# Autodesk Inventor assembly: Aluminium profile system
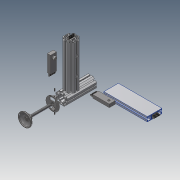
[picture p0: Inventor's stored thumbnail of the model, 180x180]
Saved by Autodesk Inventor 2015 (Build 190159000, 159)
## iProperties
Created: 2016-03-14
Part Number: Aluminium profile system
Document SubType Name: Assembly
Designer: CretelBen
Author: CretelBen
## Documents named in this file (9)
- C:\Users\CretelBen\Documents\Cretel Work\FHA2016\Booth iteration 3 - Lowered poles\Aluminium profile system\Aluminium profile system.iam
- C:\Users\CretelBen\Documents\Cretel Work\FHA2016\Booth iteration 3 - Lowered poles\Aluminium profile system\End Plate.ipt
- C:\Users\CretelBen\Documents\Cretel Work\FHA2016\Booth iteration 3 - Lowered poles\Aluminium profile system\Foot.ipt
- C:\Users\CretelBen\Documents\Cretel Work\FHA2016\Booth iteration 3 - Lowered poles\Aluminium profile system\Octagonal profile.ipt
- C:\Users\CretelBen\Documents\Cretel Work\FHA2016\Booth iteration 3 - Lowered poles\Aluminium profile system\Side bar profile.ipt
- C:\Users\CretelBen\Documents\Cretel Work\FHA2016\Booth iteration 3 - Lowered poles\Aluminium profile system\End plate set screw.ipt
- C:\Users\CretelBen\Documents\Cretel Work\FHA2016\Booth iteration 3 - Lowered poles\Aluminium profile system\Side bar connector.ipt
- C:\Users\CretelBen\Documents\Cretel Work\FHA2016\Booth iteration 3 - Lowered poles\Aluminium profile system\Octagonal profile with end connector hole.ipt
- C:\Users\CretelBen\Documents\Cretel Work\FHA2016\Booth iteration 3 - Lowered poles\Aluminium profile system\End connector.ipt
## Components (11 placed, 8 different names)
1. End Plate:1 — Mate:1, Mate:2, Mate:3, Mate:4, Mate:5, Mate:6
2. Foot:1 — Mate:1
3. Octagonal profile:1 — Mate:2, Mate:3, Mate:4
4. End plate set screw:1 — Mate:5
5. End plate set screw:2 — Mate:6
6. Side bar profile:1 — Mate:7, Mate:8, Angle:1
7. Side bar connector:1
8. Side bar connector:2 — Mate:7, Mate:8, Angle:1
9. Octagonal profile with end connector hole:1 — Mate:9, Mate:10, Angle:2
10. End connector:1
11. End connector:2 — Mate:9, Mate:10, Angle:2
## Relationships (12: Mate 10, Angle 2)
- Mate:1: End Plate:1 ↔ Foot:1
- Mate:2: End Plate:1 ↔ Octagonal profile:1
- Mate:3: End Plate:1 ↔ Octagonal profile:1
- Mate:4: End Plate:1 ↔ Octagonal profile:1
- Mate:5: End Plate:1 ↔ End plate set screw:1
- Mate:6: End Plate:1 ↔ End plate set screw:2
- Mate:7: Side bar profile:1 ↔ Side bar connector:2
- Mate:8 (0.5 mm): Side bar profile:1 ↔ Side bar connector:2
- Angle:1 (0 deg): Side bar profile:1 ↔ Side bar connector:2
- Mate:9: Octagonal profile with end connector hole:1 ↔ End connector:2
- Mate:10 (0.5 mm): Octagonal profile with end connector hole:1 ↔ End connector:2
- Angle:2 (0 deg): Octagonal profile with end connector hole:1 ↔ End connector:2
